# Autodesk Inventor assembly: Head_camera_unit_without_cover
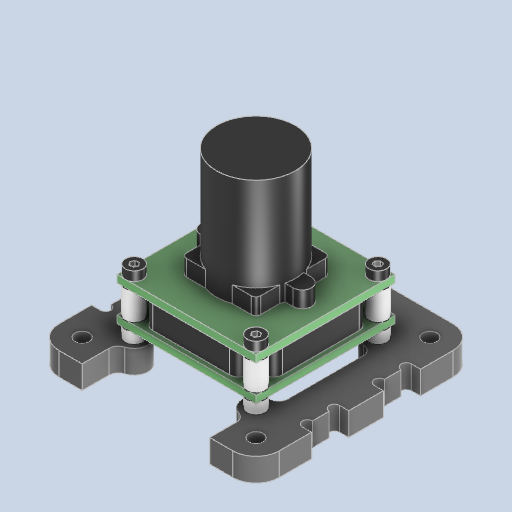
[picture p0: Inventor's stored thumbnail of the model, 512x512]
Saved by Autodesk Inventor 2022.3 (Build 263350000, 350)
## iProperties
Created: 2023-04-07
Part Number: Head_camera_unit_without_cover
Document SubType Name: Assembly
Designer: Masato Kubotera
Author: Masato Kubotera
## Documents named in this file (6)
- C:\Users\Masato\Documents\Inventor\Inventor for CIT Brains\SUSTAINA-OP - mod\UpperBody\Head\Head_camera_unit_without_cover.iam
- C:\Users\Masato\Documents\Inventor\Inventor for CIT Brains\SUSTAINA-OP - mod\ReadyMade\Camera\e-CAM50_CUNX.ipt
- C:\Users\Masato\Documents\Inventor\Inventor for CIT Brains\SUSTAINA-OP - mod\ReadyMade\Screw\FC-0215EB.ipt
- C:\Users\Masato\Documents\Inventor\Inventor for CIT Brains\SUSTAINA-OP - mod\ReadyMade\Spacer\C-2006-4.ipt
- C:\Users\Masato\Documents\Inventor\Inventor for CIT Brains\SUSTAINA-OP - mod\ReadyMade\Spacer\C-2002.5-4.ipt
- C:\Users\Masato\Documents\Inventor\Inventor for CIT Brains\SUSTAINA-OP - mod\UpperBody\Head\Head_camera_frame.iam
## Components (14 placed, 5 different names)
1. Head_camera_frame:1 [sub-assembly] — フラッシュ:1, フラッシュ:2, フラッシュ:3, 挿入:13, 挿入:14, 挿入:15, 挿入:16
2. e-CAM50_CUNX:1 — 挿入:1, 挿入:2, 挿入:3, 挿入:4, 挿入:5, 挿入:6, 挿入:7, 挿入:8, 挿入:9, 挿入:10, 挿入:11, 挿入:12
3. FC-0215EB:1 — 挿入:1
4. FC-0215EB:2 — 挿入:2
5. FC-0215EB:3 — 挿入:3
6. FC-0215EB:4 — 挿入:4
7. C-2006-4:1 — 挿入:5
8. C-2006-4:2 — 挿入:6
9. C-2006-4:3 — 挿入:7
10. C-2006-4:4 — 挿入:8
11. C-2002.5-4:1 — 挿入:9, 挿入:13
12. C-2002.5-4:2 — 挿入:10, 挿入:14
13. C-2002.5-4:3 — 挿入:11, 挿入:15
14. C-2002.5-4:4 — 挿入:12, 挿入:16
## Relationships (19: Insert 16, Flush 3)
- 挿入:1 [Insert]: e-CAM50_CUNX:1 ↔ FC-0215EB:1
- 挿入:2 [Insert]: e-CAM50_CUNX:1 ↔ FC-0215EB:2
- 挿入:3 [Insert]: e-CAM50_CUNX:1 ↔ FC-0215EB:3
- 挿入:4 [Insert]: e-CAM50_CUNX:1 ↔ FC-0215EB:4
- 挿入:5 [Insert]: e-CAM50_CUNX:1 ↔ C-2006-4:1
- 挿入:6 [Insert]: e-CAM50_CUNX:1 ↔ C-2006-4:2
- 挿入:7 [Insert]: e-CAM50_CUNX:1 ↔ C-2006-4:3
- 挿入:8 [Insert]: e-CAM50_CUNX:1 ↔ C-2006-4:4
- 挿入:9 [Insert]: e-CAM50_CUNX:1 ↔ C-2002.5-4:1
- 挿入:10 [Insert]: e-CAM50_CUNX:1 ↔ C-2002.5-4:2
- 挿入:11 [Insert]: e-CAM50_CUNX:1 ↔ C-2002.5-4:3
- 挿入:12 [Insert]: e-CAM50_CUNX:1 ↔ C-2002.5-4:4
- フラッシュ:1 [Flush]: Head_camera_frame:1
- フラッシュ:2 [Flush]: Head_camera_frame:1
- フラッシュ:3 [Flush]: Head_camera_frame:1
- 挿入:13 [Insert]: Head_camera_frame:1 ↔ C-2002.5-4:1
- 挿入:14 [Insert]: Head_camera_frame:1 ↔ C-2002.5-4:2
- 挿入:15 [Insert]: Head_camera_frame:1 ↔ C-2002.5-4:3
- 挿入:16 [Insert]: Head_camera_frame:1 ↔ C-2002.5-4:4
